# Autodesk Inventor assembly: 60T厚齿轮带铁芯_MIR
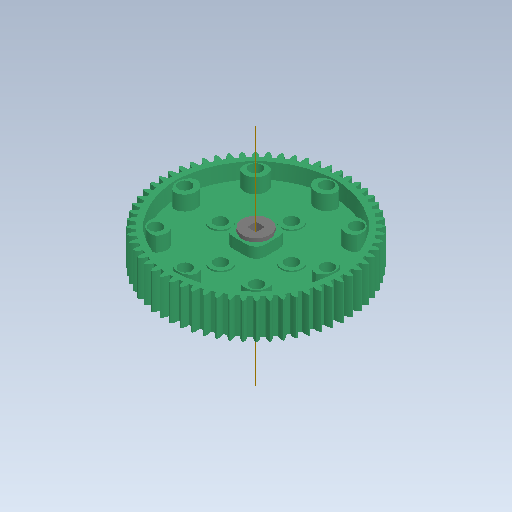
[picture p0: Inventor's stored thumbnail of the model, 512x512]
Saved by Autodesk Inventor 2020 (Build 240168000, 168)
## iProperties
Created: 2019-05-29
Part Number: 60T厚齿轮带铁芯_MIR
Document SubType Name: Assembly
Designer: 31144
Author: aresp
## Documents named in this file (3)
- C:\Users\31144\Documents\Vault\ncrCadLib\齿轮\60T厚齿轮带铁芯_MIR.iam
- C:\Users\31144\Documents\Vault\ncrCadLib\齿轮\Gear HS 60 tooth_MIR.ipt
- C:\Users\31144\Documents\Vault\ncrCadLib\齿轮\Insert HS Metal_MIR.ipt
## Components (3 placed, 2 different names)
1. Gear HS 60 tooth_MIR:1 — 配合:4, 配合:1, 配合:3, 配合:2
2. Insert HS Metal_MIR:1 — 配合:4, 配合:1, 表面齐平:1
3. Insert HS Metal_MIR:2 — 表面齐平:1, 配合:3, 配合:2
## Relationships (5: Mate 4, Flush 1)
- 配合:4 [Mate]: Gear HS 60 tooth_MIR:1 ↔ Insert HS Metal_MIR:1
- 配合:1 [Mate]: Gear HS 60 tooth_MIR:1 ↔ Insert HS Metal_MIR:1
- 表面齐平:1 [Flush]: Insert HS Metal_MIR:1 ↔ Insert HS Metal_MIR:2
- 配合:3 [Mate]: Gear HS 60 tooth_MIR:1 ↔ Insert HS Metal_MIR:2
- 配合:2 [Mate]: Gear HS 60 tooth_MIR:1 ↔ Insert HS Metal_MIR:2
